# Autodesk Inventor assembly: 知能ロボコン２
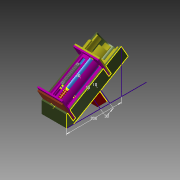
[picture p0: Inventor's stored thumbnail of the model, 180x180]
Saved by Autodesk Inventor 2013 (Build 170138000, 138)
## iProperties
Created: 2014-05-15
Part Number: 知能ロボコン２
Document SubType Name: Assembly
Designer: horumo136
Mass: 1953.83 g
Surface Area: 3092.32 cm^2
Volume: 1798.79 cm^3
Density: 1.08619 g/cm^3
Author: horumo136
## Documents named in this file (9)
- C:\Users\horumo136\Documents\知能ロボコン２.iam
- C:\Users\horumo136\Documents\知能ロボコン発射口.ipt
- C:\Users\horumo136\Documents\知能ロボコン外筒.ipt
- C:\Users\horumo136\Documents\知能ロボコンばね受け受け.ipt
- C:\Users\horumo136\Documents\知能ロボコンばね受け.ipt
- C:\Users\horumo136\Documents\知能ロボコンばね112038.ipt
- C:\Users\horumo136\Documents\知能ロボコンシリンダ.ipt
- C:\Users\horumo136\Documents\知能ロボコンラックギア.ipt
- C:\Users\horumo136\Documents\知能ロボコン発射台３.iam
## Components (8 placed, 8 different names)
1. 知能ロボコン発射口:1 — メイト:4, メイト:5, メイト:22, メイト:23
2. 知能ロボコン外筒:1 — メイト:4, メイト:5, メイト:12, メイト:13, メイト:20
3. 知能ロボコンばね受け受け:1 — メイト:8, メイト:9, メイト:10, メイト:13, メイト:20, メイト:21
4. 知能ロボコンばね受け:1 — メイト:6, メイト:7, メイト:8, メイト:9, メイト:10, メイト:12
5. 知能ロボコンばね112038:1 — メイト:6, メイト:7
6. 知能ロボコンシリンダ:1 — メイト:17
7. 知能ロボコンラックギア:1 — メイト:17
8. 知能ロボコン発射台３:1 [sub-assembly] — メイト:21, メイト:22, メイト:23
## Relationships (14: Mate 14)
- メイト:4 [Mate]: 知能ロボコン発射口:1 ↔ 知能ロボコン外筒:1
- メイト:5 [Mate]: 知能ロボコン発射口:1 ↔ 知能ロボコン外筒:1
- メイト:6 [Mate]: 知能ロボコンばね受け:1 ↔ 知能ロボコンばね112038:1
- メイト:7 [Mate]: 知能ロボコンばね受け:1 ↔ 知能ロボコンばね112038:1
- メイト:8 [Mate]: 知能ロボコンばね受け受け:1 ↔ 知能ロボコンばね受け:1
- メイト:9 [Mate]: 知能ロボコンばね受け受け:1 ↔ 知能ロボコンばね受け:1
- メイト:10 [Mate]: 知能ロボコンばね受け受け:1 ↔ 知能ロボコンばね受け:1
- メイト:12 [Mate]: 知能ロボコン外筒:1 ↔ 知能ロボコンばね受け:1
- メイト:13 [Mate]: 知能ロボコン外筒:1 ↔ 知能ロボコンばね受け受け:1
- メイト:17 [Mate]: 知能ロボコンシリンダ:1 ↔ 知能ロボコンラックギア:1
- メイト:20 [Mate]: 知能ロボコン外筒:1 ↔ 知能ロボコンばね受け受け:1
- メイト:21 [Mate]: 知能ロボコンばね受け受け:1 ↔ 知能ロボコン発射台３:1
- メイト:22 [Mate]: 知能ロボコン発射口:1 ↔ 知能ロボコン発射台３:1
- メイト:23 [Mate]: 知能ロボコン発射口:1 ↔ 知能ロボコン発射台３:1
